# Autodesk Inventor assembly: сборка_держатель_серво_брови
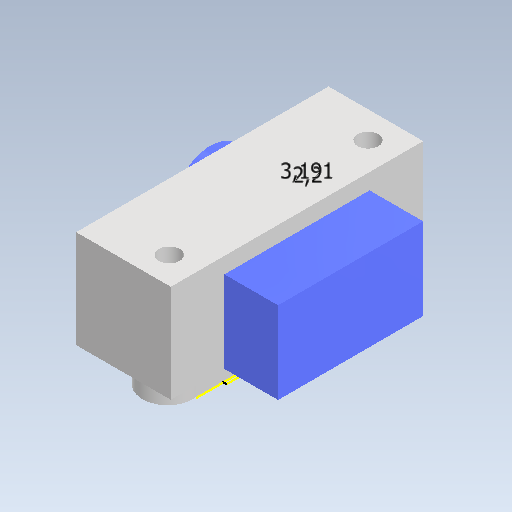
[picture p0: Inventor's stored thumbnail of the model, 512x512]
Saved by Autodesk Inventor 2020 (Build 240168000, 168)
## iProperties
Created: 2022-03-05
Part Number: сборка_держатель_серво_брови
Document SubType Name: Assembly
Designer: Администратор
Author: Администратор
## Documents named in this file (4)
- C:\Users\air13\Documents\3D\уборка\Face 2.0 full\2\сборка_держатель_серво_брови.iam
- C:\Users\air13\Documents\3D\уборка\Face 2.0 full\2\держалка_серво_бровь_нижняя.ipt
- C:\Users\air13\Documents\3D\уборка\Face 2.0 full\2\крышка_держалка_серво_брови.ipt
- C:\Users\air13\Documents\3D\уборка\Face 2.0 full\2\SERVO.ipt
## Components (3 placed, 3 different names)
1. держалка_серво_бровь_нижняя:1 — Совмещение:1, Совмещение:2
2. крышка_держалка_серво_брови:1
3. SERVO:1 — Совмещение:1, Совмещение:2
## Relationships (2: Mate 2)
- Совмещение:1 [Mate]: держалка_серво_бровь_нижняя:1 ↔ SERVO:1
- Совмещение:2 [Mate]: держалка_серво_бровь_нижняя:1 ↔ SERVO:1
